# Autodesk Inventor assembly: Assembly1TankDrive
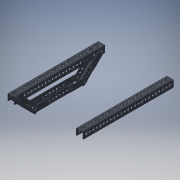
[picture p0: Inventor's stored thumbnail of the model, 180x180]
Saved by Autodesk Inventor 2016 (Build 200138000, 138)
## iProperties
Created: 2015-09-29
Part Number: Assembly1TankDrive
Document SubType Name: Assembly
Designer: phiro
Author: phiro
## Documents named in this file (5)
- C:\Users\phiro\Documents\GitHub\phi_robotics\3d-models\FTC_Tetrix_KOP_Block_Party\Assembly1TankDrive.iam
- C:\Users\phiro\Documents\GitHub\phi_robotics\3d-models\FTC_Tetrix_KOP_Block_Party\Tetrix_Kit_FTC\Autodesk Inventor Files\tetrix_c_channel-5.ipt
- C:\Users\phiro\Documents\GitHub\phi_robotics\3d-models\FTC_Tetrix_KOP_Block_Party\Tetrix_Kit_FTC\Autodesk Inventor Files\tetrix_739061_2012.ipt
- C:\Users\phiro\Documents\GitHub\phi_robotics\3d-models\FTC_Tetrix_KOP_Block_Party\Tetrix_Kit_FTC\Autodesk Inventor Files\tetrix_c_channel-2.ipt
- C:\Users\phiro\Documents\GitHub\phi_robotics\3d-models\FTC_Tetrix_KOP_Block_Party\Tetrix_Kit_FTC\Autodesk Inventor Files\tetrix_c_channel-3.ipt
## Components (13 placed, 4 different names)
1. tetrix_c_channel-5:1 — Rigid:1, Rigid:2, Rigid:4, Rigid:5
2. tetrix_c_channel-5:2
3. tetrix_739061_2012:1 — Rigid:2
4. tetrix_739061_2012:2 — Rigid:1, Rigid:3
5. tetrix_c_channel-2:1 — Rigid:3, Rigid:6, Rigid:8
6. tetrix_739061_2012:3 — Rigid:4
7. tetrix_739061_2012:4 — Rigid:5, Rotational:1
8. tetrix_c_channel-2:2 — Rotational:1, Rigid:7, Rigid:9
9. tetrix_c_channel-3:1 — Rigid:10
10. tetrix_739061_2012:5 — Rigid:7, Rigid:10
11. tetrix_739061_2012:6 — Rigid:9
12. tetrix_739061_2012:7 — Rigid:8
13. tetrix_739061_2012:8 — Rigid:6
## Relationships (11: WeldJoint 10, RevoluteJoint 1)
- Rigid:1 [WeldJoint]: tetrix_c_channel-5:1 ↔ tetrix_739061_2012:2
- Rigid:2 [WeldJoint]: tetrix_c_channel-5:1 ↔ tetrix_739061_2012:1
- Rigid:3 [WeldJoint]: tetrix_739061_2012:2 ↔ tetrix_c_channel-2:1
- Rigid:4 [WeldJoint]: tetrix_c_channel-5:1 ↔ tetrix_739061_2012:3
- Rigid:5 [WeldJoint]: tetrix_c_channel-5:1 ↔ tetrix_739061_2012:4
- Rotational:1 [RevoluteJoint]: tetrix_739061_2012:4 ↔ tetrix_c_channel-2:2
- Rigid:6 [WeldJoint]: tetrix_c_channel-2:1 ↔ tetrix_739061_2012:8
- Rigid:7 [WeldJoint]: tetrix_c_channel-2:2 ↔ tetrix_739061_2012:5
- Rigid:8 [WeldJoint]: tetrix_c_channel-2:1 ↔ tetrix_739061_2012:7
- Rigid:9 [WeldJoint]: tetrix_c_channel-2:2 ↔ tetrix_739061_2012:6
- Rigid:10 [WeldJoint]: tetrix_c_channel-3:1 ↔ tetrix_739061_2012:5
